# Autodesk Inventor assembly: Motor Mount with Motor
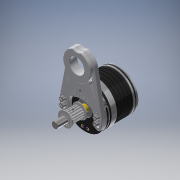
[picture p0: Inventor's stored thumbnail of the model, 180x180]
Saved by Autodesk Inventor 2019.4 (Build 234330000, 330)
## iProperties
Created: 2019-03-01
Part Number: Motor Mount with Motor
Document SubType Name: Assembly
Designer: Petar
Mass: 37.7633 g
Surface Area: 102.459 cm^2
Volume: 12.7696 cm^3
Density: 2.95729 g/cm^3
Author: Petar
## Documents named in this file (14)
- D:\OMG\E-Board\CAD\Inventor\Mechanical Components\Assemblies\Motor Mount (225-ABS) with Motor.iam
- D:\OMG\E-Board\CAD\Inventor\Mechanical Components\Motor Mount\Ring Mount\Mount Ring - ABS.ipt
- D:\OMG\E-Board\CAD\Inventor\Electric Motor\Turnigy SK8 5045.iam
- D:\OMG\E-Board\CAD\Inventor\Mechanical Components\Motor Mount\Holder Mount\Motor Holder v3 - 225 - ABS.ipt
- D:\OMG\E-Board\CAD\Inventor\Mechanical Components\Assemblies\Motor Mount with Motor\Design Accelerator\Bolted Connection5.iam
- D:\OMG\E-Board\CAD\Inventor\Mechanical Components\Assemblies\Motor Mount with Motor\Design Accelerator\Bolted Connection6.iam
- D:\OMG\E-Board\CAD\Inventor\Mechanical Components\Assemblies\Motor Mount with Motor\Design Accelerator\Bolted Connection7.iam
- D:\OMG\E-Board\CAD\Inventor\Mechanical Components\Assemblies\Motor Mount with Motor\Design Accelerator\Bolted Connection8.iam
- D:\OMG\E-Board\CAD\Inventor\Mechanical Components\Assemblies\Motor Mount with Motor\AIP\FEA\ct0fs6600.fins
- D:\OMG\E-Board\CAD\Inventor\Mechanical Components\Assemblies\Motor Mount with Motor\AIP\FEA\ct0fs660w.fsat
- D:\OMG\E-Board\CAD\Inventor\Mechanical Components\Assemblies\Motor Mount with Motor\AIP\FEA\ct0fs660w.ftes
- D:\OMG\E-Board\CAD\Inventor\Mechanical Components\Assemblies\Motor Mount with Motor\AIP\FEA\ct0fs660w.fwiz
- D:\OMG\E-Board\CAD\Inventor\Mechanical Components\Assemblies\Motor Mount with Motor\AIP\FEA\ct0fs66e8.fmsh
- D:\OMG\E-Board\CAD\Inventor\Mechanical Components\Assemblies\Motor Mount with Motor\AIP\FEA\ct0fs66e9.fres
## Components (7 placed, 4 different names)
1. Mount Ring - ABS:1 — Rigid:1
2. Motor Holder v3 - 225 - ABS:1 — Rigid:1, Rigid:2, Mate:9, Mate:11, Mate:13, Mate:15
3. Turnigy SK8 5045:1 [sub-assembly] — Rigid:2, Mate:10, Mate:12, Mate:14, Mate:16
4. Bolted Connection:1 [sub-assembly] — Mate:9, Mate:10
5. Bolted Connection:2 [sub-assembly] — Mate:11, Mate:12
6. Bolted Connection:3 [sub-assembly] — Mate:13, Mate:14
7. Bolted Connection:4 [sub-assembly] — Mate:15, Mate:16
## Relationships (10: Mate 8, WeldJoint 2)
- Rigid:1 [WeldJoint]: Mount Ring - ABS:1 ↔ Motor Holder v3 - 225 - ABS:1
- Rigid:2 [WeldJoint]: Motor Holder v3 - 225 - ABS:1 ↔ Turnigy SK8 5045:1
- Mate:9: Motor Holder v3 - 225 - ABS:1 ↔ Bolted Connection:1
- Mate:10: Turnigy SK8 5045:1 ↔ Bolted Connection:1
- Mate:11: Motor Holder v3 - 225 - ABS:1 ↔ Bolted Connection:2
- Mate:12: Turnigy SK8 5045:1 ↔ Bolted Connection:2
- Mate:13: Motor Holder v3 - 225 - ABS:1 ↔ Bolted Connection:3
- Mate:14: Turnigy SK8 5045:1 ↔ Bolted Connection:3
- Mate:15: Motor Holder v3 - 225 - ABS:1 ↔ Bolted Connection:4
- Mate:16: Turnigy SK8 5045:1 ↔ Bolted Connection:4
## Named parameters: sa_3 = 338.445, sa_4 = 15900, sa_0 = 33800
note: some values were not read from the file. Shown as the stored number, unit unknown: "sa_3", "sa_4", "sa_0".
